# Autodesk Inventor assembly: Onderbeen
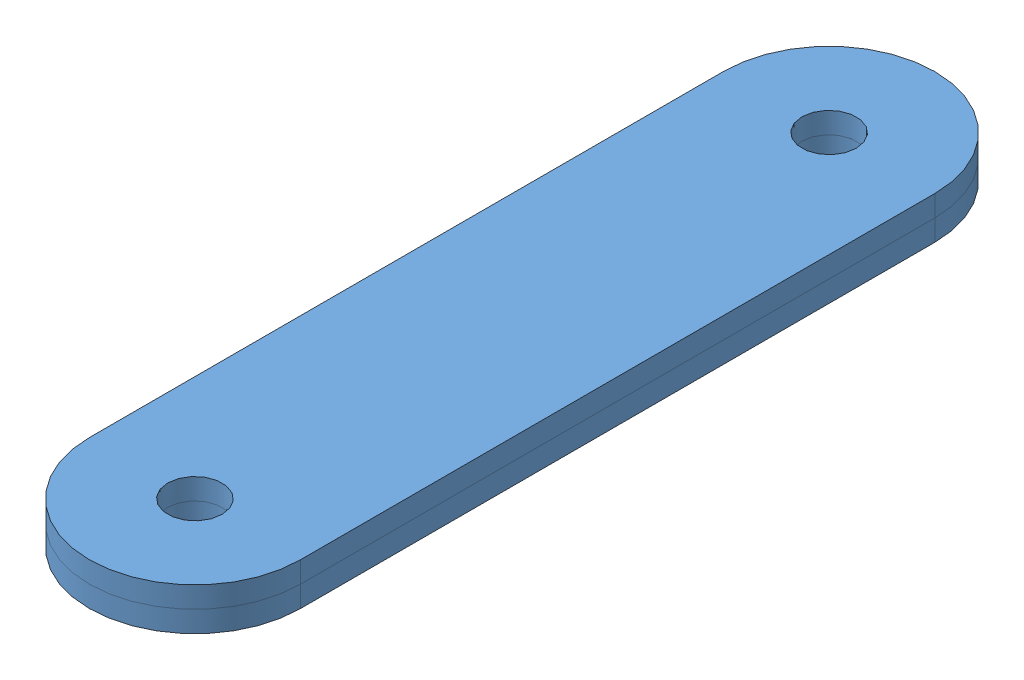
[picture p0: shaded view drawn from the part files that the assembly names]
Saved by Autodesk Inventor 2015 (Build 190159000, 159)
## iProperties
Created: 2015-12-21
Part Number: Onderbeen
Document SubType Name: Assembly
Designer: david
Author: david
## Documents named in this file (2)
- Z:\gip\Inventor\generatie 7\Beenen\onderbeen\Onderbeen.iam
- Z:\gip\Inventor\generatie 7\Beenen\onderbeen\onderbeen.ipt
## Components (2 placed, 1 different names)
1. onderbeen:1 — Mate:1, Mate:2, Flush:1
2. onderbeen:2 — Mate:1, Mate:2, Flush:1
## Relationships (3: Mate 2, Flush 1)
- Mate:1: onderbeen:1 ↔ onderbeen:2
- Mate:2: onderbeen:1 ↔ onderbeen:2
- Flush:1: onderbeen:1 ↔ onderbeen:2
